# Autodesk Inventor assembly: Link3ver2
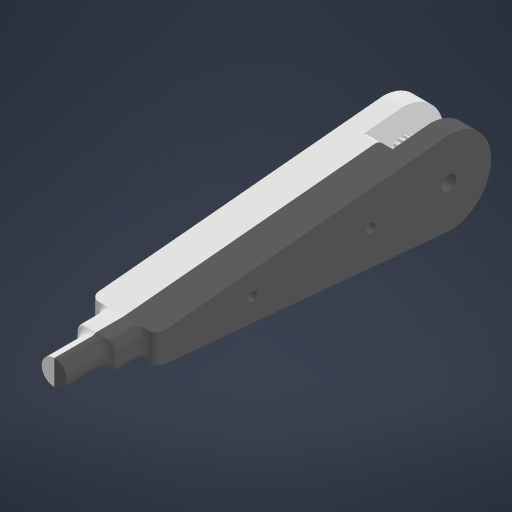
[picture p0: Inventor's stored thumbnail of the model, 512x512]
Saved by Autodesk Inventor 2023 (Build 270158000, 158)
## iProperties
Created: 2023-09-14
Part Number: Link3ver2
Document SubType Name: Assembly
Designer: philo
Author: philo
## Documents named in this file (2)
- C:\Users\philo\OneDrive\Desktop\HK1-2024\TT ROBOT\02_3D_design_new\Link3ver2.iam
- C:\Users\philo\OneDrive\Desktop\HK1-2024\TT ROBOT\02_3D_design_new\Part2.ipt
## Components (2 placed, 1 different names)
1. Part2:1 — Mate:1, Mate:2, Mate:3
2. Part2:2 — Mate:1, Mate:2, Mate:3
## Relationships (3: Mate 3)
- Mate:1: Part2:1 ↔ Part2:2
- Mate:2: Part2:1 ↔ Part2:2
- Mate:3: Part2:1 ↔ Part2:2
